# Autodesk Inventor assembly: 61weller
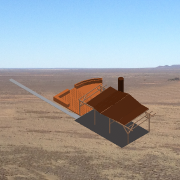
[picture p0: Inventor's stored thumbnail of the model, 180x180]
Saved by Autodesk Inventor 2013 SP2 (Build 170200200, 200)
## iProperties
Created: 2014-01-02
Part Number: 61weller
Document SubType Name: Assembly
Designer: ddeboer
Author: ddeboer
## Documents named in this file (10)
- C:\Users\Dave\Desktop\house-cad\61weller.iam
- C:\Users\Dave\Desktop\house-cad\plat.ipt
- C:\Users\Dave\Desktop\house-cad\patio.iam
- C:\Users\Dave\Desktop\house-cad\sidewalkBack.ipt
- C:\Users\Dave\Desktop\house-cad\2by4by16.ipt
- C:\Users\Dave\Desktop\house-cad\2by4by12.ipt
- C:\Users\Dave\Desktop\house-cad\tree.ipt
- C:\Users\Dave\Desktop\house-cad\wrapAround.ipt
- C:\Users\Dave\Desktop\house-cad\bench.ipt
- C:\Users\Dave\Desktop\house-cad\planter.ipt
## Components (64 placed, 9 different names)
1. plat:1 — Insert:1
2. patio:1 [sub-assembly] — Insert:1, Mate:1, Flush:1, Mate:2, Flush:2, Mate:5, Flush:5
3. sidewalkBack:1 — Mate:1, Flush:1, Mate:3
4. tree:1 — Mate:5, Flush:5
5. wrapAround:1 — Mate:6, Flush:6, Mate:8, Flush:10, Flush:11
6. bench:1 — Mate:7, Flush:8, Flush:9
7. planter:1 — Mate:8, Flush:10, Flush:11
8. 2by4by16:1 — Mate:2, Mate:3, Flush:2, Mate:4, Flush:3, Flush:4
9. 2by4by16:2
10. 2by4by16:3
11. 2by4by16:4
12. 2by4by16:5
13. 2by4by16:6
14. 2by4by16:7
15. 2by4by16:8
16. 2by4by16:9
17. 2by4by12:1 — Mate:4, Flush:3, Flush:4
18. 2by4by12:2
19. 2by4by12:3
20. 2by4by12:4
21. 2by4by12:5
22. 2by4by12:6
23. 2by4by12:7
24. 2by4by12:8
25. 2by4by12:9
26. 2by4by12:10
27. 2by4by12:11
28. 2by4by12:12
29. 2by4by12:13 — Flush:6
30. 2by4by12:14
31. 2by4by12:15
32. 2by4by12:16
33. 2by4by12:17
34. 2by4by12:18
35. 2by4by12:19
36. 2by4by12:20
37. 2by4by12:21
38. 2by4by12:22
39. 2by4by12:23
40. 2by4by12:24
41. 2by4by12:25
42. 2by4by12:26 — Flush:9
43. 2by4by12:27
44. 2by4by12:28
45. 2by4by12:29
46. 2by4by12:30
47. 2by4by12:31
48. 2by4by12:32
49. 2by4by12:33
50. 2by4by12:34
51. 2by4by12:35
52. 2by4by12:36
53. 2by4by12:37 — Mate:6
54. 2by4by12:38
55. 2by4by12:39
56. 2by4by12:40
57. 2by4by12:41
58. 2by4by12:42
59. 2by4by12:43
60. 2by4by12:44
61. 2by4by12:45
62. 2by4by12:46
63. 2by4by12:47
64. 2by4by12:48 — Mate:7, Flush:8
## Component patterns: (9 elements, first: 2by4by16:1), (48 elements, first: 2by4by12:1)
## Relationships (19: Flush 10, Mate 8, Insert 1)
- Insert:1: plat:1 ↔ patio:1
- Mate:1: patio:1 ↔ sidewalkBack:1
- Flush:1 (-355.6 mm): patio:1 ↔ sidewalkBack:1
- Mate:2: patio:1 ↔ 2by4by16:1
- Mate:3: sidewalkBack:1 ↔ 2by4by16:1
- Flush:2 (-152.4 mm): patio:1 ↔ 2by4by16:1
- Mate:4: 2by4by16:1 ↔ 2by4by12:1
- Flush:3: 2by4by16:1 ↔ 2by4by12:1
- Flush:4: 2by4by16:1 ↔ 2by4by12:1
- Mate:5 (1524 mm): patio:1 ↔ tree:1
- Flush:5 (1016 mm): patio:1 ↔ tree:1
- Mate:6: wrapAround:1 ↔ 2by4by12:37
- Flush:6: wrapAround:1 ↔ 2by4by12:13
- Mate:7: bench:1 ↔ 2by4by12:48
- Flush:8: bench:1 ↔ 2by4by12:48
- Flush:9: bench:1 ↔ 2by4by12:26
- Mate:8: wrapAround:1 ↔ planter:1
- Flush:10: wrapAround:1 ↔ planter:1
- Flush:11: wrapAround:1 ↔ planter:1
